# Autodesk Inventor assembly: Ensamblaje d
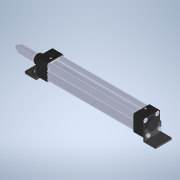
[picture p0: Inventor's stored thumbnail of the model, 180x180]
Saved by Autodesk Inventor 2021 (Build 250183000, 183)
## iProperties
Created: 2021-02-23
Part Number: Ensamblaje d
Document SubType Name: Assembly
Designer: jalej
Author: jalej
Sending System: SolidWorks 2020
Last Author: marte
Last Saved: 2021-10-26
## Documents named in this file (15)
- C:\Users\jalej\OneDrive - UNIVERSIDAD NACIONAL AUTÓNOMA DE MÉXICO\Desktop\Documents-OneDrive\10mo_SEM\SCADA\Proyecto1\HMI_Proyecto1\Cilindros neumáticos\Cilindro de doble efecto\Imported Components\Ensamblaje d.iam
- C:\Users\jalej\OneDrive - UNIVERSIDAD NACIONAL AUTÓNOMA DE MÉXICO\Desktop\Documents-OneDrive\10mo_SEM\SCADA\Proyecto1\HMI_Proyecto1\Cilindros neumáticos\Cilindro de doble efecto\Imported Components\Ensamblaje d.ipt
- C:\Users\jalej\OneDrive - UNIVERSIDAD NACIONAL AUTÓNOMA DE MÉXICO\Desktop\Documents-OneDrive\10mo_SEM\SCADA\Proyecto1\HMI_Proyecto1\Cilindros neumáticos\Cilindro de doble efecto\Imported Components\Ensamblaje d_Predeterminado.ipt
- C:\Users\jalej\OneDrive - UNIVERSIDAD NACIONAL AUTÓNOMA DE MÉXICO\Desktop\Documents-OneDrive\10mo_SEM\SCADA\Proyecto1\HMI_Proyecto1\Cilindros neumáticos\Cilindro de doble efecto\Imported Components\Ensamblaje d_Predeterminado_1.ipt
- C:\Users\jalej\OneDrive - UNIVERSIDAD NACIONAL AUTÓNOMA DE MÉXICO\Desktop\Documents-OneDrive\10mo_SEM\SCADA\Proyecto1\HMI_Proyecto1\Cilindros neumáticos\Cilindro de doble efecto\Imported Components\Ensamblaje d_Predeterminado_9.ipt
- C:\Users\jalej\OneDrive - UNIVERSIDAD NACIONAL AUTÓNOMA DE MÉXICO\Desktop\Documents-OneDrive\10mo_SEM\SCADA\Proyecto1\HMI_Proyecto1\Cilindros neumáticos\Cilindro de doble efecto\Imported Components\Ensamblaje d_Predeterminado_10.ipt
- C:\Users\jalej\OneDrive - UNIVERSIDAD NACIONAL AUTÓNOMA DE MÉXICO\Desktop\Documents-OneDrive\10mo_SEM\SCADA\Proyecto1\HMI_Proyecto1\Cilindros neumáticos\Cilindro de doble efecto\Imported Components\Ensamblaje d_Predeterminado_11.ipt
- C:\Users\jalej\OneDrive - UNIVERSIDAD NACIONAL AUTÓNOMA DE MÉXICO\Desktop\Documents-OneDrive\10mo_SEM\SCADA\Proyecto1\HMI_Proyecto1\Cilindros neumáticos\Cilindro de doble efecto\Imported Components\Ensamblaje d_Predeterminado_12.ipt
- C:\Users\jalej\OneDrive - UNIVERSIDAD NACIONAL AUTÓNOMA DE MÉXICO\Desktop\Documents-OneDrive\10mo_SEM\SCADA\Proyecto1\HMI_Proyecto1\Cilindros neumáticos\Cilindro de doble efecto\Imported Components\Ensamblaje d_Predeterminado_13.ipt
- C:\Users\jalej\OneDrive - UNIVERSIDAD NACIONAL AUTÓNOMA DE MÉXICO\Desktop\Documents-OneDrive\10mo_SEM\SCADA\Proyecto1\HMI_Proyecto1\Cilindros neumáticos\Cilindro de doble efecto\Imported Components\Ensamblaje d_Predeterminado_14.ipt
- C:\Users\jalej\OneDrive - UNIVERSIDAD NACIONAL AUTÓNOMA DE MÉXICO\Desktop\Documents-OneDrive\10mo_SEM\SCADA\Proyecto1\HMI_Proyecto1\Cilindros neumáticos\Cilindro de doble efecto\Imported Components\Ensamblaje d_Predeterminado_15.ipt
- C:\Users\jalej\OneDrive - UNIVERSIDAD NACIONAL AUTÓNOMA DE MÉXICO\Desktop\Documents-OneDrive\10mo_SEM\SCADA\Proyecto1\HMI_Proyecto1\Cilindros neumáticos\Cilindro de doble efecto\Imported Components\Ensamblaje d_Predeterminado_16.ipt
- C:\Users\jalej\OneDrive - UNIVERSIDAD NACIONAL AUTÓNOMA DE MÉXICO\Desktop\Documents-OneDrive\10mo_SEM\SCADA\Proyecto1\HMI_Proyecto1\Cilindros neumáticos\Cilindro de doble efecto\Imported Components\Ensamblaje d_Predeterminado_17.ipt
- C:\Users\jalej\OneDrive - UNIVERSIDAD NACIONAL AUTÓNOMA DE MÉXICO\Desktop\Documents-OneDrive\10mo_SEM\SCADA\Proyecto1\HMI_Proyecto1\Cilindros neumáticos\Cilindro de doble efecto\Imported Components\Ensamblaje d_Predeterminado_18.ipt
- C:\Users\jalej\OneDrive - UNIVERSIDAD NACIONAL AUTÓNOMA DE MÉXICO\Desktop\Documents-OneDrive\10mo_SEM\SCADA\Proyecto1\HMI_Proyecto1\Cilindros neumáticos\Cilindro de doble efecto\Vástago.ipt
## Components (29 placed, 14 different names)
1. Camisa:1 — Coincidencia:4, Coincidencia:5
2. Tapa Trasera:2 — Coincidencia:5
3. Tapa Delantera:1 — Coincidencia:2, Coincidencia:4
4. Junta Estática:1
5. Tornillo:1
6. Tornillo:2
7. Tornillo:3
8. Tornillo:5
9. Tornillo:6
10. Tornillo:8
11. Tornillo:9
12. Tornillo:11
13. Anillo_Rascador:1 — Coincidencia:3, Coincidencia:8
14. Sello:1
15. Soportes de pie:1
16. Soportes de pie:2
17. Sello:2
18. Junta_Estatica2:2
19. Junta_Estatica2:4
20. Junta Estática:2
21. Tornillo de ajuste de amortiguamiento:1
22. Tornillo de ajuste de amortiguamiento:2
23. DIN-912 - M5x10:1
24. DIN-912 - M5x10:3
25. DIN-912 - M5x10:4
26. DIN-912 - M5x10:5
27. Cabeza del pistón:1 — Coincidencia:6, Coincidencia:7
28. Tuerca:1 — De rotación:1, Coincidencia:6, Coincidencia:8
29. Vástago:1 — De rotación:1, Coincidencia:2, Coincidencia:3, Coincidencia:7
## Relationships (8: Mate 7, RevoluteJoint 1)
- De rotación:1 [RevoluteJoint]: Tuerca:1 ↔ Vástago:1
- Coincidencia:2 [Mate]: Tapa Delantera:1 ↔ Vástago:1
- Coincidencia:3 [Mate]: Anillo_Rascador:1 ↔ Vástago:1
- Coincidencia:4 [Mate]: Camisa:1 ↔ Tapa Delantera:1
- Coincidencia:5 [Mate]: Camisa:1 ↔ Tapa Trasera:2
- Coincidencia:6 [Mate]: Cabeza del pistón:1 ↔ Tuerca:1
- Coincidencia:7 [Mate]: Cabeza del pistón:1 ↔ Vástago:1
- Coincidencia:8 [Mate]: Anillo_Rascador:1 ↔ Tuerca:1
